# Autodesk Inventor assembly: Assembly1
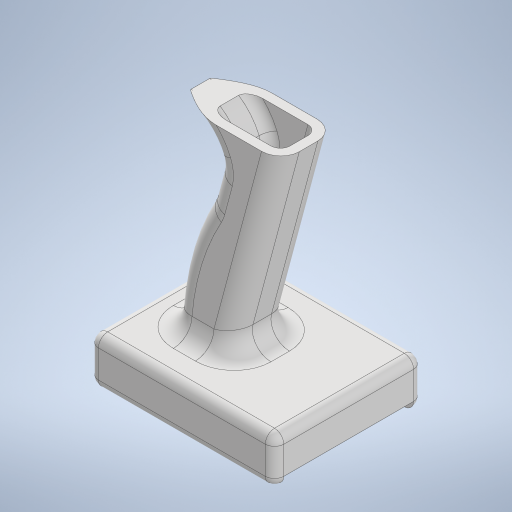
[picture p0: Inventor's stored thumbnail of the model, 512x512]
Saved by Autodesk Inventor 2023.2 (Build 272271030, 271C)
## iProperties
Created: 2023-03-18
Part Number: Assembly1
Document SubType Name: Assembly
Designer: oktay
Author: oktay
## Documents named in this file (3)
- C:\Users\oktay\Desktop\kumanda\Assembly1.iam
- C:\Users\oktay\Desktop\kumanda\kumanda alt.ipt
- C:\Users\oktay\Desktop\kumanda\battery-holder-aasize-1-5v-4-1.snapshot.3\Battery Holder.iam
## Components (2 placed, 2 different names)
1. kumanda alt:1 — Mate:1
2. Battery Holder:1 [sub-assembly] — Mate:1
## Relationships (1: Mate 1)
- Mate:1: kumanda alt:1 ↔ Battery Holder:1
